# Autodesk Inventor assembly: ForeArm
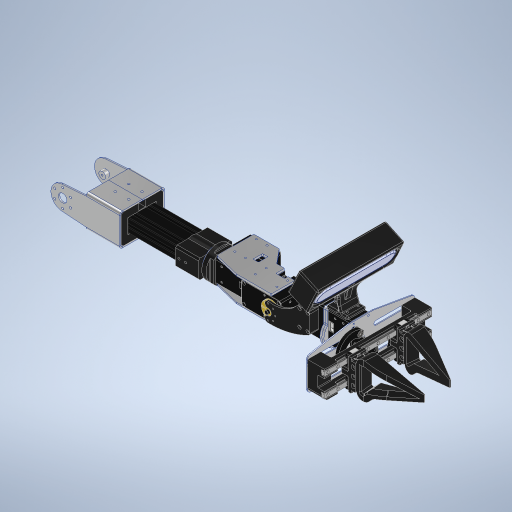
[picture p0: Inventor's stored thumbnail of the model, 512x512]
Saved by Autodesk Inventor 2024.3 (Build 283343010, 343A)
## iProperties
Created: 2025-05-20
Part Number: ForeArm
Document SubType Name: Assembly
Designer: kshau
Mass: 2677.24 g
Surface Area: 4102.22 cm^2
Volume: 921.382 cm^3
Density: 2.90568 g/cm^3
Author: kshau
## Documents named in this file (21)
- C:\Users\kshau\Documents\inventor\Create_ViperX\Create_ViperX_ALOHA\ForeArm_Component\ForeArm.iam
- C:\Users\kshau\Documents\inventor\Create_ViperX\Create_ViperX_ALOHA\ForeArm_Component\fore_parameter.ipt
- C:\Users\kshau\Documents\inventor\Create_ViperX\Create_ViperX_ALOHA\ForeArm_Component\framefixpart1_forearm.ipt
- C:\Users\kshau\Documents\inventor\Create_ViperX\Create_ViperX_ALOHA\ForeArm_Component\connectpart1.ipt
- C:\Users\kshau\Documents\inventor\Create_ViperX\Create_ViperX_ALOHA\Actuator\XM,H,D-540.N101.I101\XM,H,D-540.N101.I101\XM,H,D-540.N101.I101.ipt
- C:\Users\kshau\Documents\inventor\Create_ViperX\Create_ViperX_ALOHA\ForeArm_Component\connectplate1.ipt
- C:\Users\kshau\Documents\inventor\Create_ViperX\Create_ViperX_ALOHA\Actuator\XM,H-430_idler\XM,H-430_idler\XM,H-430_idler.iam
- C:\Users\kshau\Documents\inventor\Create_ViperX\Create_ViperX_ALOHA\NessesaryParts\HFSB5-2040-140_STEP_AP203_20250629\HFSB5-2040-140\HFSB5-2040-140\HFSB5-2040-140.ipt
- C:\Users\kshau\Documents\inventor\Create_ViperX\Create_ViperX_ALOHA\ForeArm_Component\cameramount.ipt
- C:\Users\kshau\Documents\inventor\Create_ViperX\Create_ViperX_ALOHA\NessesaryParts\Intel Realsense D455\Intel Realsense D455\Intel Realsense D455.iam
- C:\Users\kshau\Documents\inventor\Create_ViperX\Create_ViperX_ALOHA\ForeArm_Component\connectplate2.ipt
- C:\Users\kshau\Documents\inventor\Create_ViperX\Create_ViperX_ALOHA\ForeArm_Component\servoplate1_forR0.ipt
- C:\Users\kshau\Documents\inventor\Create_ViperX\Create_ViperX_ALOHA\ForeArm_Component\servoplate2_forR0.ipt
- C:\Users\kshau\Documents\inventor\Create_ViperX\Create_ViperX_ALOHA\ForeArm_Component\connectplate4.ipt
- C:\Users\kshau\Documents\inventor\Create_ViperX\Create_ViperX_ALOHA\ForeArm_Component\connectplate3.ipt
- C:\Users\kshau\Documents\inventor\Create_ViperX\Create_ViperX_ALOHA\ForeArm_Component\shortshaft2.ipt
- C:\Users\kshau\Documents\inventor\Create_ViperX\Create_ViperX_ALOHA\ForeArm_Component\connectplate5.ipt
- C:\Users\kshau\Documents\inventor\Create_ViperX\Create_ViperX_ALOHA\ForeArm_Component\connectpart2.ipt
- C:\Users\kshau\Documents\inventor\Create_ViperX\Create_ViperX_ALOHA\ForeArm_Component\connectpart3.ipt
- C:\Users\kshau\Documents\inventor\Create_ViperX\Create_ViperX_ALOHA\ForeArm_Component\connectpart3_MIR1.ipt
- C:\Users\kshau\Documents\inventor\Create_ViperX\Create_ViperX_ALOHA\ILOHA_hand\iloha_hand_ver2.iam
## Components (21 placed, 20 different names)
1. fore_parameter:1
2. servoplate1_forR0:1 — 回転:1, 回転:2
3. framefixpart1_forearm:1 — 回転:1, 回転:2, 回転:3, 回転:4, フラッシュ:1, フラッシュ:2, メイト:5, 回転:25, 回転:26
4. servoplate2_forR0:1 — 回転:3, 回転:4, 回転:35
5. connectplate5:1 — 回転:5, 回転:6, メイト:1, メイト:2, 回転:7, 回転:8
6. connectpart1:1 — 回転:5, 回転:6, フラッシュ:1, フラッシュ:2, メイト:5
7. connectpart2:1 — メイト:1, メイト:2, メイト:6
8. XM,H,D-540.N101.I101:1 — 回転:7, 回転:8, 回転:9, 回転:10, 回転:11, 回転:12, メイト:6
9. connectplate1:1 — 回転:9, 回転:10, 回転:13
10. connectplate2:1 — 回転:11, 回転:12, 回転:14
11. XM,H,D-540.N101.I101:2 — 回転:13, 回転:14, 回転:15, 回転:16, 回転:36, 回転:37
12. connectpart3:1 — 回転:15, 回転:16
13. XM,H-430_idler:1 [sub-assembly] — メイト:3, メイト:4, フラッシュ:3, 回転:38, 回転:39
14. connectplate3:1 — メイト:3, メイト:4, 回転:23, 回転:24, フラッシュ:3
15. connectplate4:1 — 回転:23, 回転:24, 回転:40, 回転:41
16. HFSB5-2040-140:1 — 回転:25, 回転:26
17. cameramount:1 — 回転:29, 回転:30, 回転:42, 回転:43
18. Intel Realsense D455:1 [sub-assembly] — 回転:29, 回転:30
19. shortshaft2:1 — 回転:35
20. connectpart3_MIR1:1 — 回転:36, 回転:37, 回転:38, 回転:39
21. iloha_hand_ver2:1 [sub-assembly] — 回転:40, 回転:41, 回転:42, 回転:43
## Relationships (40: RevoluteJoint 31, Mate 6, Flush 3)
- 回転:1 [RevoluteJoint]: servoplate1_forR0:1 ↔ framefixpart1_forearm:1
- 回転:2 [RevoluteJoint]: servoplate1_forR0:1 ↔ framefixpart1_forearm:1
- 回転:3 [RevoluteJoint]: framefixpart1_forearm:1 ↔ servoplate2_forR0:1
- 回転:4 [RevoluteJoint]: framefixpart1_forearm:1 ↔ servoplate2_forR0:1
- 回転:5 [RevoluteJoint]: connectplate5:1 ↔ connectpart1:1
- 回転:6 [RevoluteJoint]: connectplate5:1 ↔ connectpart1:1
- メイト:1 [Mate]: connectplate5:1 ↔ connectpart2:1
- メイト:2 [Mate]: connectplate5:1 ↔ connectpart2:1
- 回転:7 [RevoluteJoint]: connectplate5:1 ↔ XM,H,D-540.N101.I101:1
- 回転:8 [RevoluteJoint]: connectplate5:1 ↔ XM,H,D-540.N101.I101:1
- フラッシュ:1 [Flush]: framefixpart1_forearm:1 ↔ connectpart1:1
- フラッシュ:2 [Flush]: framefixpart1_forearm:1 ↔ connectpart1:1
- 回転:9 [RevoluteJoint]: XM,H,D-540.N101.I101:1 ↔ connectplate1:1
- 回転:10 [RevoluteJoint]: XM,H,D-540.N101.I101:1 ↔ connectplate1:1
- 回転:11 [RevoluteJoint]: XM,H,D-540.N101.I101:1 ↔ connectplate2:1
- 回転:12 [RevoluteJoint]: XM,H,D-540.N101.I101:1 ↔ connectplate2:1
- 回転:13 [RevoluteJoint]: connectplate1:1 ↔ XM,H,D-540.N101.I101:2
- 回転:14 [RevoluteJoint]: connectplate2:1 ↔ XM,H,D-540.N101.I101:2
- 回転:15 [RevoluteJoint]: XM,H,D-540.N101.I101:2 ↔ connectpart3:1
- 回転:16 [RevoluteJoint]: XM,H,D-540.N101.I101:2 ↔ connectpart3:1
- メイト:3 [Mate]: XM,H-430_idler:1 ↔ connectplate3:1
- メイト:4 [Mate]: XM,H-430_idler:1 ↔ connectplate3:1
- 回転:23 [RevoluteJoint]: connectplate3:1 ↔ connectplate4:1
- 回転:24 [RevoluteJoint]: connectplate3:1 ↔ connectplate4:1
- フラッシュ:3 [Flush]: XM,H-430_idler:1 ↔ connectplate3:1
- メイト:5 [Mate] (75 mm): framefixpart1_forearm:1 ↔ connectpart1:1
- 回転:25 [RevoluteJoint]: framefixpart1_forearm:1 ↔ HFSB5-2040-140:1
- 回転:26 [RevoluteJoint]: framefixpart1_forearm:1 ↔ HFSB5-2040-140:1
- メイト:6 [Mate]: connectpart2:1 ↔ XM,H,D-540.N101.I101:1
- 回転:29 [RevoluteJoint]: cameramount:1 ↔ Intel Realsense D455:1
- 回転:30 [RevoluteJoint]: cameramount:1 ↔ Intel Realsense D455:1
- 回転:35 [RevoluteJoint]: servoplate2_forR0:1 ↔ shortshaft2:1
- 回転:36 [RevoluteJoint]: XM,H,D-540.N101.I101:2 ↔ connectpart3_MIR1:1
- 回転:37 [RevoluteJoint]: XM,H,D-540.N101.I101:2 ↔ connectpart3_MIR1:1
- 回転:38 [RevoluteJoint]: XM,H-430_idler:1 ↔ connectpart3_MIR1:1
- 回転:39 [RevoluteJoint]: XM,H-430_idler:1 ↔ connectpart3_MIR1:1
- 回転:40 [RevoluteJoint]: connectplate4:1 ↔ iloha_hand_ver2:1
- 回転:41 [RevoluteJoint]: connectplate4:1 ↔ iloha_hand_ver2:1
- 回転:42 [RevoluteJoint]: cameramount:1 ↔ iloha_hand_ver2:1
- 回転:43 [RevoluteJoint]: cameramount:1 ↔ iloha_hand_ver2:1
